# Autodesk Inventor assembly: Panel Back
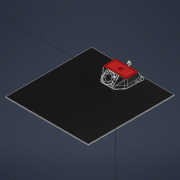
[picture p0: Inventor's stored thumbnail of the model, 180x180]
Saved by Autodesk Inventor 2022.2 (Build 262287010, 287A)
## iProperties
Created: 2022-03-16
Part Number: Panel Back
Document SubType Name: Assembly
Designer: sleib
Author: sleib
## Documents named in this file (8)
- C:\Users\sleib\Projekte\Voron-2\CAD\Inventor\Panel Back.iam
- C:\Users\sleib\Projekte\Voron-2\CAD\Inventor\Foamtape Side.ipt
- C:\Users\sleib\Projekte\Voron-2\CAD\Inventor\Panel Back.ipt
- C:\Users\sleib\Projekte\Voron-2\CAD\Inventor\Exhaust Grill.ipt
- Exhaust Grill.ipt
- C:\Users\sleib\Projekte\Voron-2\CAD\Inventor\Exhaust Filter-Unit.iam
- C:\Users\sleib\Projekte\Voron-2\CAD\Inventor\M3x8 SHCS.ipt
- C:\Users\sleib\Projekte\Voron-2\CAD\Inventor\BMP280 Holder.ipt
## Components (9 placed, 6 different names)
1. Panel Back:1 — Passend:1, Passend:2, Fluchtend:1, Passend:3, Passend:4, Passend:5, Passend:6, Passend:7, Passend:8, Passend:13
2. Foamtape Side:1 — Passend:1, Passend:2, Fluchtend:1
3. Exhaust Grill:1 — Passend:3, Passend:4, Passend:5, Passend:11, Passend:12
4. Exhaust Filter-Unit:1 [sub-assembly] — Passend:6, Passend:7, Passend:8, Passend:9, Passend:10, Passend:17, Passend:18
5. M3x8 SHCS:1 — Passend:9, Passend:12
6. M3x8 SHCS:2 — Passend:10, Passend:11
7. BMP280 Holder:1 — Passend:13, Passend:19, Passend:20, Passend:21, Passend:22
8. M3x8 SHCS:3 — Passend:17, Passend:20, Passend:21
9. M3x8 SHCS:4 — Passend:18, Passend:19, Passend:22
## Relationships (20: Mate 19, Flush 1)
- Passend:1 [Mate]: Panel Back:1 ↔ Foamtape Side:1
- Passend:2 [Mate]: Panel Back:1 ↔ Foamtape Side:1
- Fluchtend:1 [Flush]: Panel Back:1 ↔ Foamtape Side:1
- Passend:3 [Mate]: Panel Back:1 ↔ Exhaust Grill:1
- Passend:4 [Mate]: Panel Back:1 ↔ Exhaust Grill:1
- Passend:5 [Mate]: Panel Back:1 ↔ Exhaust Grill:1
- Passend:6 [Mate]: Panel Back:1 ↔ Exhaust Filter-Unit:1
- Passend:7 [Mate]: Panel Back:1 ↔ Exhaust Filter-Unit:1
- Passend:8 [Mate]: Panel Back:1 ↔ Exhaust Filter-Unit:1
- Passend:9 [Mate]: Exhaust Filter-Unit:1 ↔ M3x8 SHCS:1
- Passend:10 [Mate]: Exhaust Filter-Unit:1 ↔ M3x8 SHCS:2
- Passend:11 [Mate]: Exhaust Grill:1 ↔ M3x8 SHCS:2
- Passend:12 [Mate]: Exhaust Grill:1 ↔ M3x8 SHCS:1
- Passend:13 [Mate]: Panel Back:1 ↔ BMP280 Holder:1
- Passend:17 [Mate]: Exhaust Filter-Unit:1 ↔ M3x8 SHCS:3
- Passend:18 [Mate]: Exhaust Filter-Unit:1 ↔ M3x8 SHCS:4
- Passend:19 [Mate]: BMP280 Holder:1 ↔ M3x8 SHCS:4
- Passend:20 [Mate]: BMP280 Holder:1 ↔ M3x8 SHCS:3
- Passend:21 [Mate]: BMP280 Holder:1 ↔ M3x8 SHCS:3
- Passend:22 [Mate]: BMP280 Holder:1 ↔ M3x8 SHCS:4
